# Autodesk Inventor assembly: total asssembly
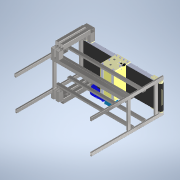
[picture p0: Inventor's stored thumbnail of the model, 180x180]
Saved by Autodesk Inventor 2022.2 (Build 262287010, 287A)
## iProperties
_SolveAssemblyDoc: Frame Generator Solve Assembly
_Version: 25.0.0
Created: 2022-02-23
Part Number: total asssembly
Document SubType Name: Assembly
Designer: ONG
Author: ONG
## Documents named in this file (7)
- C:\Users\ONG\Documents\INVENTOR DESIGN\音箱\total asssembly.iam
- C:\Users\ONG\Documents\INVENTOR DESIGN\音箱\frame.ipt
- C:\Users\ONG\Downloads\belt conveyour\ARCANE 300х1000\Frame\Frame 1645576523614.iam
- C:\Users\ONG\Downloads\belt conveyour\ARCANE 300х1000.iam
- C:\Users\ONG\Documents\INVENTOR DESIGN\音箱\stand one part.ipt
- C:\Users\ONG\Documents\INVENTOR DESIGN\音箱\total asssembly\Frame\Frame 1645577982344.iam
- C:\Users\ONG\Documents\INVENTOR DESIGN\音箱\OBJECT.ipt
## Components (9 placed, 6 different names)
1. frame:1
2. Frame 1645576523614:1 [sub-assembly] — Mate:2, Mate:7, Flush:3, Mate:8, Mate:12, Mate:13, Flush:7
3. ARCANE 300х1000:1 [sub-assembly] — Mate:2, Rigid:1
4. stand one part:1 — Flush:6, Mate:13, Mate:14
5. stand one part:2 — Flush:5, Mate:11, Mate:12
6. stand one part:3 — Mate:7, Mate:9, Flush:4
7. stand one part:4 — Flush:3, Mate:8, Mate:10
8. Frame 1645577982344:1 [sub-assembly] — Mate:9, Flush:4, Mate:10, Flush:5, Mate:11, Flush:6, Mate:14, Flush:7
9. OBJECT:1 — Rigid:1
## Relationships (15: Mate 9, Flush 5, WeldJoint 1)
- Mate:2: Frame 1645576523614:1 ↔ ARCANE 300х1000:1
- Mate:7: Frame 1645576523614:1 ↔ stand one part:3
- Flush:3 (-5 mm): Frame 1645576523614:1 ↔ stand one part:4
- Mate:8: Frame 1645576523614:1 ↔ stand one part:4
- Mate:9: stand one part:3 ↔ Frame 1645577982344:1
- Flush:4: stand one part:3 ↔ Frame 1645577982344:1
- Mate:10: stand one part:4 ↔ Frame 1645577982344:1
- Flush:5: stand one part:2 ↔ Frame 1645577982344:1
- Mate:11: stand one part:2 ↔ Frame 1645577982344:1
- Mate:12: Frame 1645576523614:1 ↔ stand one part:2
- Flush:6: stand one part:1 ↔ Frame 1645577982344:1
- Mate:13: Frame 1645576523614:1 ↔ stand one part:1
- Mate:14: stand one part:1 ↔ Frame 1645577982344:1
- Flush:7: Frame 1645576523614:1 ↔ Frame 1645577982344:1
- Rigid:1 [WeldJoint]: ARCANE 300х1000:1 ↔ OBJECT:1
